# Autodesk Inventor assembly: ASY GBK 3220 central wall shield 5
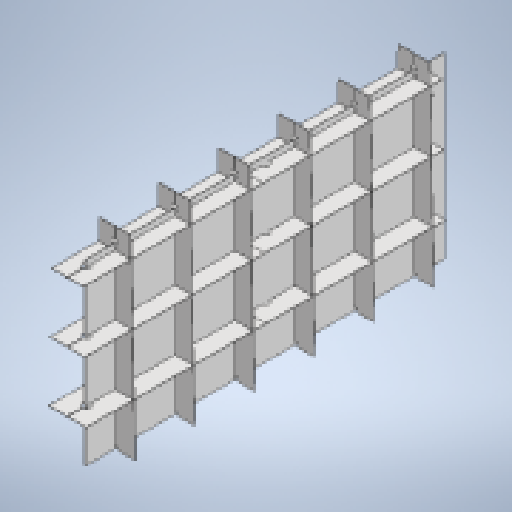
[picture p0: Inventor's stored thumbnail of the model, 512x512]
Saved by Autodesk Inventor 2026 (Build 300175000, 175)
## iProperties
Created: 2026-05-19
Part Number: ASY GBK 3220 central wall shield 5
Document SubType Name: Assembly
Designer: pokla
Mass: 152628 g
Surface Area: 99280.6 cm^2
Volume: 19443.1 cm^3
Density: 7.85 g/cm^3
Author: admin
## Documents named in this file (8)
- C:\Users\pokla\Documents\Inventor\GBK-Gubkinskiy\ASY GBK 3220 central wall shield 5.iam
- C:\Users\pokla\Documents\Inventor\GBK-Gubkinskiy\GBK 0101 main rib.ipt
- C:\Users\pokla\Documents\Inventor\GBK-Gubkinskiy\GBK 3225 shield 5.ipt
- C:\Users\pokla\Documents\Inventor\GBK-Gubkinskiy\GBK 3212 central second rib_CPY.ipt
- GBK 3212 central second rib_CPY.ipt
- C:\Users\pokla\Documents\Inventor\GBK-Gubkinskiy\GBK 3214 stringer 4.ipt
- C:\Users\pokla\Documents\Inventor\GBK-Gubkinskiy\GBK 3215 stringer 5.ipt
- C:\Users\pokla\Documents\Inventor\GBK-Gubkinskiy\GBK 3216 stringer 6.ipt
## Components (25 placed, 5 different names)
1. GBK 3214 stringer 4:1 — Жесткий:1, Жесткий:10
2. GBK 3215 stringer 5:1 — Жесткий:2, Жесткий:11
3. GBK 3216 stringer 6:1 — Жесткий:3, Жесткий:12
4. GBK 3214 stringer 4:2 — Жесткий:6, Жесткий:7
5. GBK 3215 stringer 5:2 — Жесткий:5, Жесткий:8
6. GBK 3216 stringer 6:2 — Жесткий:4, Жесткий:9
7. GBK 3224 shield 4:1 — Заподлицо:6, Совмещение:7, Совмещение:8, Совмещение:6, Заподлицо:8, Заподлицо:7, Совмещение:5
8. GBK 3214 stringer 4:3 — Жесткий:7
9. GBK 3215 stringer 5:3 — Жесткий:8
10. GBK 3216 stringer 6:3 — Жесткий:9
11. GBK 3214 stringer 4:4 — Жесткий:10
12. GBK 3215 stringer 5:4 — Жесткий:11
13. GBK 3216 stringer 6:4 — Жесткий:12
14. GBK 3212 central second rib_CPY:1 — Заподлицо:8, Заподлицо:7, Совмещение:5, Заподлицо:4, Совмещение:5, Жесткий:4, Жесткий:5, Жесткий:6
15. GBK 3212 central second rib_CPY:2 — Совмещение:6, Совмещение:6, Заподлицо:4, Жесткий:3, Жесткий:2, Жесткий:1
16. GBK 3212 central second rib_CPY:3
17. GBK 3212 central second rib_CPY:4
18. GBK 3212 central second rib_CPY:5
19. GBK 3212 central second rib_CPY:6
20. GBK 3212 central second rib_CPY:7
21. GBK 3212 central second rib_CPY:8
22. GBK 3212 central second rib_CPY:9
23. GBK 3212 central second rib_CPY:10
24. GBK 3212 central second rib_CPY:11
25. GBK 3212 central second rib_CPY:12
## Component patterns: (6 elements, first: GBK 3212 central second rib_CPY:1 + GBK 3212 central second rib_CPY:2)
## Relationships (22: WeldJoint 12, Mate 6, Flush 4)
- Заподлицо:6 [Flush]: GBK 3224 shield 4:1
- Совмещение:7 [Mate]: GBK 3224 shield 4:1
- Совмещение:8 [Mate]: GBK 3224 shield 4:1
- Совмещение:6 [Mate]: GBK 3224 shield 4:1 ↔ GBK 3212 central second rib_CPY:2
- Совмещение:6 [Mate]: GBK 3212 central second rib_CPY:2
- Заподлицо:8 [Flush] (250 mm): GBK 3224 shield 4:1 ↔ GBK 3212 central second rib_CPY:1
- Заподлицо:7 [Flush]: GBK 3224 shield 4:1 ↔ GBK 3212 central second rib_CPY:1
- Совмещение:5 [Mate]: GBK 3224 shield 4:1 ↔ GBK 3212 central second rib_CPY:1
- Заподлицо:4 [Flush]: GBK 3212 central second rib_CPY:1 ↔ GBK 3212 central second rib_CPY:2
- Совмещение:5 [Mate]: GBK 3212 central second rib_CPY:1
- Жесткий:3 [WeldJoint] (4 mm): GBK 3216 stringer 6:1 ↔ GBK 3212 central second rib_CPY:2
- Жесткий:2 [WeldJoint] (4 mm): GBK 3215 stringer 5:1 ↔ GBK 3212 central second rib_CPY:2
- Жесткий:1 [WeldJoint] (4 mm): GBK 3214 stringer 4:1 ↔ GBK 3212 central second rib_CPY:2
- Жесткий:4 [WeldJoint] (4 mm): GBK 3216 stringer 6:2 ↔ GBK 3212 central second rib_CPY:1
- Жесткий:5 [WeldJoint] (4 mm): GBK 3215 stringer 5:2 ↔ GBK 3212 central second rib_CPY:1
- Жесткий:6 [WeldJoint] (4 mm): GBK 3214 stringer 4:2 ↔ GBK 3212 central second rib_CPY:1
- Жесткий:7 [WeldJoint]: GBK 3214 stringer 4:2 ↔ GBK 3214 stringer 4:3
- Жесткий:8 [WeldJoint]: GBK 3215 stringer 5:2 ↔ GBK 3215 stringer 5:3
- Жесткий:9 [WeldJoint]: GBK 3216 stringer 6:2 ↔ GBK 3216 stringer 6:3
- Жесткий:10 [WeldJoint]: GBK 3214 stringer 4:1 ↔ GBK 3214 stringer 4:4
- Жесткий:11 [WeldJoint]: GBK 3215 stringer 5:1 ↔ GBK 3215 stringer 5:4
- Жесткий:12 [WeldJoint]: GBK 3216 stringer 6:1 ↔ GBK 3216 stringer 6:4
## Named parameters: основание_длина_нижнего = 196 mm, основание_длина_верхнего = 96 mm, стрингер_глубина_1 = 186.70056 mm, стрингер_глубина_2 = 175.35977 mm, стрингер_глубина_3 = 164.01899 mm, стрингер_глубина_4 = 152.6782 mm, стрингер_глубина_5 = 141.33742 mm, стрингер_глубина_6 = 129.99663 mm, стрингер_глубина_7 = 118.65585 mm, стрингер_глубина_8 = 107.31507 mm, Лист_ширина = 1480 mm, ребро_усилителей = 60 mm, паз_под_стрингер_глубина = 70 mm, паз_под_стрингер_толщина = 5 mm, отступ_от_пола_до_первого_стрингера = 410 mm, шаг_стрингеров = 500 mm, радиус_выреза_под_сварку = 30 mm, нахлест_шпангоутов_1_2 = 150 mm, нахлест_шпангоутов_2_3 = 120 mm, Стрингер_длина = 1490 mm, Лист_длина = 2980 mm, Шаг_шпангоутов = 496.66667 mm
